# Autodesk Inventor assembly: A2017_T4_01
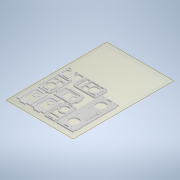
[picture p0: Inventor's stored thumbnail of the model, 180x180]
Saved by Autodesk Inventor 2020 (Build 240168000, 168)
## iProperties
Created: 2021-08-27
Part Number: A2017_T4_01
Document SubType Name: Assembly
Designer: Masato
Author: Masato
## Documents named in this file (7)
- C:\Inventor\OpenPlatform_ver3_0\cam\A2017_T4_01.iam
- C:\Inventor\OpenPlatform_ver3_0\cam\Disposable_Board.ipt
- C:\Inventor\OpenPlatform_ver3_0\UpperBody\Trunk\Trunk_neck_Upper_frame.ipt
- C:\Inventor\OpenPlatform_ver3_0\UpperBody\Trunk\Trunk_shoulder_frame_.ipt
- C:\Inventor\OpenPlatform_ver3_0\UpperBody\Trunk\Trunk_shoulder_frame_MIR.ipt
- C:\Inventor\OpenPlatform_ver3_0\UpperBody\Trunk\Trunk_waisit_frame_.ipt
- C:\Inventor\OpenPlatform_ver3_0\UpperBody\Trunk\Trunk_servo_bottom_frame.ipt
## Components (8 placed, 6 different names)
1. Disposable_Board:1 — メイト:2, メイト:1, フラッシュ:1, フラッシュ:2, メイト:4, メイト:6, メイト:7, メイト:8, メイト:9, メイト:10, フラッシュ:3, フラッシュ:6, フラッシュ:8, フラッシュ:10, メイト:19, フラッシュ:11, フラッシュ:12
2. Trunk_neck_Upper_frame:1 — メイト:6, メイト:15, フラッシュ:10, メイト:16, メイト:24
3. Trunk_shoulder_frame_:1 — メイト:4, フラッシュ:3, メイト:23, メイト:25, メイト:27
4. Trunk_shoulder_frame_MIR:1 — メイト:19, メイト:26, メイト:27
5. Trunk_waisit_frame_:1 — メイト:7, フラッシュ:8, メイト:16, メイト:26
6. Trunk_servo_bottom_frame:1 — メイト:10, フラッシュ:11, フラッシュ:12, メイト:22, メイト:23
7. Trunk_servo_bottom_frame:2 — メイト:9, メイト:24, メイト:25
8. Trunk_servo_bottom_frame:3 — メイト:8, フラッシュ:6, メイト:15, メイト:22
## Relationships (25: Mate 17, Flush 8)
- メイト:2 [Mate]: Disposable_Board:1
- メイト:1 [Mate]: Disposable_Board:1
- フラッシュ:1 [Flush]: Disposable_Board:1
- フラッシュ:2 [Flush]: Disposable_Board:1
- メイト:4 [Mate]: Disposable_Board:1 ↔ Trunk_shoulder_frame_:1
- メイト:6 [Mate]: Disposable_Board:1 ↔ Trunk_neck_Upper_frame:1
- メイト:7 [Mate]: Disposable_Board:1 ↔ Trunk_waisit_frame_:1
- メイト:8 [Mate]: Disposable_Board:1 ↔ Trunk_servo_bottom_frame:3
- メイト:9 [Mate]: Disposable_Board:1 ↔ Trunk_servo_bottom_frame:2
- メイト:10 [Mate]: Disposable_Board:1 ↔ Trunk_servo_bottom_frame:1
- フラッシュ:3 [Flush] (2.5 mm): Disposable_Board:1 ↔ Trunk_shoulder_frame_:1
- フラッシュ:6 [Flush] (2.5 mm): Disposable_Board:1 ↔ Trunk_servo_bottom_frame:3
- フラッシュ:8 [Flush] (2.5 mm): Disposable_Board:1 ↔ Trunk_waisit_frame_:1
- メイト:15 [Mate] (2.5 mm): Trunk_neck_Upper_frame:1 ↔ Trunk_servo_bottom_frame:3
- フラッシュ:10 [Flush] (2.5 mm): Disposable_Board:1 ↔ Trunk_neck_Upper_frame:1
- メイト:16 [Mate] (2.5 mm): Trunk_neck_Upper_frame:1 ↔ Trunk_waisit_frame_:1
- メイト:19 [Mate]: Disposable_Board:1 ↔ Trunk_shoulder_frame_MIR:1
- フラッシュ:11 [Flush] (2.5 mm): Disposable_Board:1 ↔ Trunk_servo_bottom_frame:1
- フラッシュ:12 [Flush] (2.5 mm): Disposable_Board:1 ↔ Trunk_servo_bottom_frame:1
- メイト:22 [Mate] (2.5 mm): Trunk_servo_bottom_frame:1 ↔ Trunk_servo_bottom_frame:3
- メイト:23 [Mate] (2.5 mm): Trunk_shoulder_frame_:1 ↔ Trunk_servo_bottom_frame:1
- メイト:24 [Mate] (2.5 mm): Trunk_neck_Upper_frame:1 ↔ Trunk_servo_bottom_frame:2
- メイト:25 [Mate] (2.5 mm): Trunk_shoulder_frame_:1 ↔ Trunk_servo_bottom_frame:2
- メイト:26 [Mate] (2.5 mm): Trunk_shoulder_frame_MIR:1 ↔ Trunk_waisit_frame_:1
- メイト:27 [Mate] (2.5 mm): Trunk_shoulder_frame_:1 ↔ Trunk_shoulder_frame_MIR:1
